# Autodesk Inventor assembly: field_and_shooter
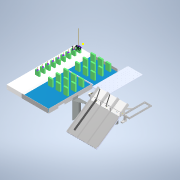
[picture p0: Inventor's stored thumbnail of the model, 180x180]
Saved by Autodesk Inventor 2022 (Build 260153000, 153)
## iProperties
Created: 2021-09-13
Part Number: field_and_shooter
Document SubType Name: Assembly
Designer: yuto6
Author: yuto6
## Documents named in this file (11)
- C:\Users\yuto6\Box\Public_Share\キャチロボバトルコンテスト2021\CAD\catchrobo_hardware\assy-shooter\field_and_shooter.iam
- C:\Users\yuto6\Box\Public_Share\キャチロボバトルコンテスト2021\CAD\catchrobo_hardware\field\aassy-blue_side.iam
- C:\Users\yuto6\Box\Public_Share\キャチロボバトルコンテスト2021\CAD\catchrobo_hardware\assy-shooter\s-assy-shooter_frame.iam
- C:\Users\yuto6\Box\Public_Share\キャチロボバトルコンテスト2021\CAD\catchrobo_hardware\assy-shooter\s-assy-shooter_unit.iam
- C:\Users\yuto6\Box\Public_Share\キャチロボバトルコンテスト2021\CAD\catchrobo_hardware\assy-shooter\s_base1_2.ipt
- C:\Users\yuto6\Box\Public_Share\キャチロボバトルコンテスト2021\CAD\catchrobo_hardware\assy-shooter\s_carbon_plate1.ipt
- C:\Users\yuto6\Box\Public_Share\キャチロボバトルコンテスト2021\CAD\catchrobo_hardware\assy-shooter\s_base2.ipt
- C:\Users\yuto6\Box\Public_Share\キャチロボバトルコンテスト2021\CAD\catchrobo_hardware\assy-shooter\s-assy-sorter.iam
- C:\Users\yuto6\Box\Public_Share\キャチロボバトルコンテスト2021\CAD\catchrobo_hardware\assy-shooter\s_base4_2.ipt
- C:\Users\yuto6\Box\Public_Share\キャチロボバトルコンテスト2021\CAD\catchrobo_hardware\assy-shooter\s-assy-shooter_pulley.iam
- C:\Users\yuto6\Box\Public_Share\キャチロボバトルコンテスト2021\CAD\catchrobo_hardware\assy-shooter\s_base8.ipt
## Components (14 placed, 10 different names)
1. aassy-blue_side:1 [sub-assembly] — メイト:1, フラッシュ:1, フラッシュ:2, フラッシュ:3, メイト:2
2. s-assy-shooter_frame:1 [sub-assembly] — メイト:1, フラッシュ:1, メイト:3, フラッシュ:4, フラッシュ:8, メイト:14, フラッシュ:9, メイト:15, フラッシュ:10, メイト:16, メイト:24, フラッシュ:13
3. s-assy-shooter_unit:1 [sub-assembly] — フラッシュ:2, フラッシュ:3, メイト:2, メイト:5, フラッシュ:5, メイト:6, メイト:17, メイト:18, メイト:23, フラッシュ:12
4. s_base1_2:1 — メイト:3, フラッシュ:4, メイト:18
5. s_carbon_plate1:1 — メイト:5, フラッシュ:5, メイト:6, メイト:7, フラッシュ:6, メイト:8, メイト:11, メイト:12, メイト:13
6. s_carbon_plate1:2 — メイト:9, フラッシュ:7, メイト:10, メイト:19, メイト:20, メイト:21, フラッシュ:11, メイト:22
7. s_base2:1 — メイト:7, フラッシュ:6, メイト:8, メイト:9, フラッシュ:7, メイト:10
8. s-assy-sorter:1 [sub-assembly] — メイト:11, メイト:12, メイト:13
9. s_base1_2:2 — フラッシュ:10, メイト:16, メイト:20
10. s_base1_2:3 — フラッシュ:9, メイト:15, メイト:19
11. s_base1_2:4 — フラッシュ:8, メイト:14, メイト:17
12. s_base4_2:1 — メイト:21, フラッシュ:11, メイト:22
13. s-assy-shooter_pulley:1 [sub-assembly] — メイト:23, フラッシュ:12
14. s_base8:1 — メイト:24, フラッシュ:13
## Relationships (36: Mate 23, Flush 13)
- メイト:1 [Mate]: aassy-blue_side:1 ↔ s-assy-shooter_frame:1
- フラッシュ:1 [Flush] (60 mm): aassy-blue_side:1 ↔ s-assy-shooter_frame:1
- フラッシュ:2 [Flush]: aassy-blue_side:1 ↔ s-assy-shooter_unit:1
- フラッシュ:3 [Flush]: aassy-blue_side:1 ↔ s-assy-shooter_unit:1
- メイト:2 [Mate] (2 mm): aassy-blue_side:1 ↔ s-assy-shooter_unit:1
- メイト:3 [Mate]: s-assy-shooter_frame:1 ↔ s_base1_2:1
- フラッシュ:4 [Flush]: s-assy-shooter_frame:1 ↔ s_base1_2:1
- メイト:5 [Mate]: s-assy-shooter_unit:1 ↔ s_carbon_plate1:1
- フラッシュ:5 [Flush]: s-assy-shooter_unit:1 ↔ s_carbon_plate1:1
- メイト:6 [Mate]: s-assy-shooter_unit:1 ↔ s_carbon_plate1:1
- メイト:7 [Mate]: s_carbon_plate1:1 ↔ s_base2:1
- フラッシュ:6 [Flush]: s_carbon_plate1:1 ↔ s_base2:1
- メイト:8 [Mate]: s_carbon_plate1:1 ↔ s_base2:1
- メイト:9 [Mate]: s_carbon_plate1:2 ↔ s_base2:1
- フラッシュ:7 [Flush]: s_carbon_plate1:2 ↔ s_base2:1
- メイト:10 [Mate]: s_carbon_plate1:2 ↔ s_base2:1
- メイト:11 [Mate]: s_carbon_plate1:1 ↔ s-assy-sorter:1
- メイト:12 [Mate]: s_carbon_plate1:1 ↔ s-assy-sorter:1
- メイト:13 [Mate]: s_carbon_plate1:1 ↔ s-assy-sorter:1
- フラッシュ:8 [Flush]: s-assy-shooter_frame:1 ↔ s_base1_2:4
- メイト:14 [Mate]: s-assy-shooter_frame:1 ↔ s_base1_2:4
- フラッシュ:9 [Flush]: s-assy-shooter_frame:1 ↔ s_base1_2:3
- メイト:15 [Mate]: s-assy-shooter_frame:1 ↔ s_base1_2:3
- フラッシュ:10 [Flush]: s-assy-shooter_frame:1 ↔ s_base1_2:2
- メイト:16 [Mate]: s-assy-shooter_frame:1 ↔ s_base1_2:2
- メイト:17 [Mate]: s-assy-shooter_unit:1 ↔ s_base1_2:4
- メイト:18 [Mate]: s-assy-shooter_unit:1 ↔ s_base1_2:1
- メイト:19 [Mate]: s_carbon_plate1:2 ↔ s_base1_2:3
- メイト:20 [Mate]: s_carbon_plate1:2 ↔ s_base1_2:2
- メイト:21 [Mate]: s_carbon_plate1:2 ↔ s_base4_2:1
- フラッシュ:11 [Flush]: s_carbon_plate1:2 ↔ s_base4_2:1
- メイト:22 [Mate]: s_carbon_plate1:2 ↔ s_base4_2:1
- メイト:23 [Mate]: s-assy-shooter_unit:1 ↔ s-assy-shooter_pulley:1
- フラッシュ:12 [Flush] (5 mm): s-assy-shooter_unit:1 ↔ s-assy-shooter_pulley:1
- メイト:24 [Mate]: s-assy-shooter_frame:1 ↔ s_base8:1
- フラッシュ:13 [Flush]: s-assy-shooter_frame:1 ↔ s_base8:1
